# Autodesk Inventor assembly: gusset
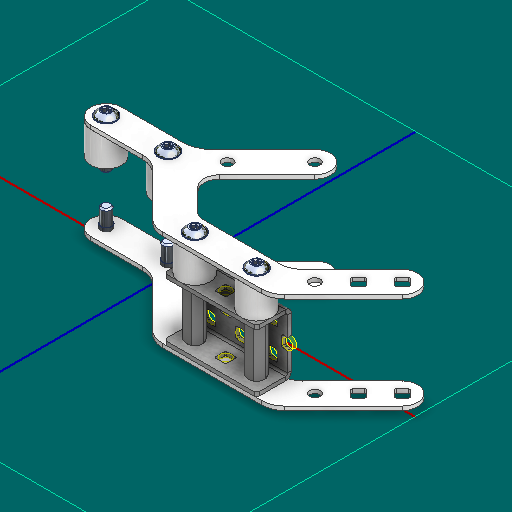
[picture p0: Inventor's stored thumbnail of the model, 512x512]
Saved by Autodesk Inventor 2025 (Build 290162000, 162)
## iProperties
Created: 2024-08-17
Part Number: gusset
Document SubType Name: Assembly
Designer: averey
Author: averey
## Documents named in this file (11)
- C:\Users\avere\vex_robotics_high_stakes\hardware\cad\ATLAS\chassis\drive_pod\gusset.iam
- C:\Users\avere\vex_robotics_high_stakes\hardware\cad\ATLAS\chassis\drive_pod\custom_parts\join_gusset.ipt
- C:\Users\avere\vex_robotics_high_stakes\hardware\cad\VEX-CAD-Inventor\Motion\Spacers\Spacer Nylon .500 OD\NSpacer White .500 OD x .500.ipt
- C:\Users\avere\vex_robotics_high_stakes\hardware\cad\VEX-CAD-Inventor\Motion\Spacers\Spacer Nylon .500 OD.ipt
- C:\Users\avere\vex_robotics_high_stakes\hardware\cad\VEX-CAD-Inventor\Structure\C Channel\Aluminum 1x2x1\Alu C 1x2x1x3.ipt
- C:\Users\avere\vex_robotics_high_stakes\hardware\cad\VEX-CAD-Inventor\Structure\Standoff\Standoff .875.ipt
- C:\Users\avere\vex_robotics_high_stakes\hardware\cad\VEX-CAD-Inventor\Structure\Standoff.ipt
- C:\Users\avere\vex_robotics_high_stakes\hardware\cad\VEX-CAD-Inventor\Structure\Hardware\Screw Steel - Star\SScrew Star Smooth .750.ipt
- C:\Users\avere\vex_robotics_high_stakes\hardware\cad\VEX-CAD-Inventor\Structure\Hardware\Screw Steel - Star.ipt
- C:\Users\avere\vex_robotics_high_stakes\hardware\cad\VEX-CAD-Inventor\Structure\Hardware\Screw Shoulder Robosource\SScrew Shoulder Smooth .375 x .12.ipt
- C:\Users\avere\vex_robotics_high_stakes\hardware\cad\VEX-CAD-Inventor\Structure\Hardware\Screw Shoulder Robosource.ipt
## Components (17 placed, 6 different names)
1. join_gusset:1 — Insert:1, Mate:1, Insert:15, Insert:17, Insert:24, Insert:26
2. join_gusset:2 — Insert:1, Mate:1, Insert:5, Insert:7, Insert:13, Insert:14, Insert:21, Insert:23, Insert:27, Insert:28
3. NSpacer White .500 OD x .500:4 — Insert:5, Insert:8
4. NSpacer White .500 OD x .500:5 — Insert:7, Mate:2
5. Alu C 1x2x1x3:1 — Insert:8, Mate:2, Insert:9, Insert:10
6. Standoff .875:1 — Insert:9
7. Standoff .875:2 — Insert:10
8. SScrew Star Smooth .750:1 — Insert:14
9. SScrew Star Smooth .750:2 — Insert:13
10. SScrew Shoulder Smooth .375 x .12:1 — Insert:15
11. SScrew Shoulder Smooth .375 x .12:2 — Insert:17
12. SScrew Star Smooth .750:4 — Insert:23
13. SScrew Star Smooth .750:6 — Insert:21
14. SScrew Shoulder Smooth .375 x .12:4 — Insert:24
15. SScrew Shoulder Smooth .375 x .12:6 — Insert:26
16. NSpacer White .500 OD x .500:6 — Insert:27
17. NSpacer White .500 OD x .500:7 — Insert:28
## Relationships (18: Insert 16, Mate 2)
- Insert:1 (38.1 mm): join_gusset:1 ↔ join_gusset:2
- Mate:1: join_gusset:1 ↔ join_gusset:2
- Insert:5: join_gusset:2 ↔ NSpacer White .500 OD x .500:4
- Insert:7: join_gusset:2 ↔ NSpacer White .500 OD x .500:5
- Insert:8: NSpacer White .500 OD x .500:4 ↔ Alu C 1x2x1x3:1
- Mate:2: NSpacer White .500 OD x .500:5 ↔ Alu C 1x2x1x3:1
- Insert:9: Alu C 1x2x1x3:1 ↔ Standoff .875:1
- Insert:10: Alu C 1x2x1x3:1 ↔ Standoff .875:2
- Insert:13: join_gusset:2 ↔ SScrew Star Smooth .750:2
- Insert:14: join_gusset:2 ↔ SScrew Star Smooth .750:1
- Insert:15: join_gusset:1 ↔ SScrew Shoulder Smooth .375 x .12:1
- Insert:17: join_gusset:1 ↔ SScrew Shoulder Smooth .375 x .12:2
- Insert:21: join_gusset:2 ↔ SScrew Star Smooth .750:6
- Insert:23: join_gusset:2 ↔ SScrew Star Smooth .750:4
- Insert:24: join_gusset:1 ↔ SScrew Shoulder Smooth .375 x .12:4
- Insert:26: join_gusset:1 ↔ SScrew Shoulder Smooth .375 x .12:6
- Insert:27: join_gusset:2 ↔ NSpacer White .500 OD x .500:6
- Insert:28: join_gusset:2 ↔ NSpacer White .500 OD x .500:7
